# Autodesk Inventor assembly: frame assembly
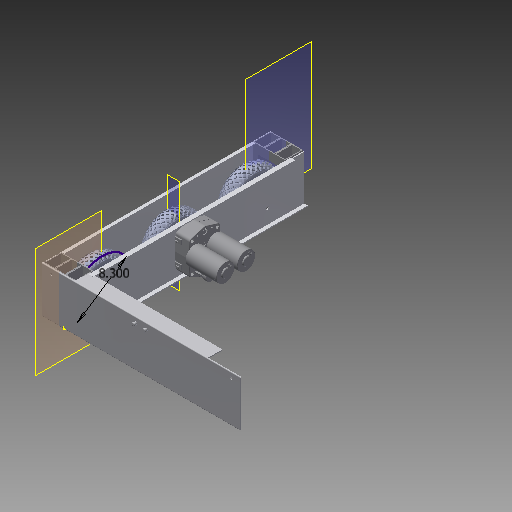
[picture p0: Inventor's stored thumbnail of the model, 512x512]
Saved by Autodesk Inventor 2017 (Build 210142000, 142)
## iProperties
Created: 2019-01-15
Part Number: frame assembly
Document SubType Name: Assembly
Designer: S346795925
Author: S346795925
## Documents named in this file (13)
- P:\frc-season-2019-deep-space-1\Robot\Robot\frame assembly.iam
- P:\frc-season-2019-deep-space-1\Robot\Robot\Frame - outside rail.ipt
- P:\frc-season-2019-deep-space-1\Robot\Robot\am-3936 Aluminum 8IN Pneumatic 500IN Hex Bore Wheel.iam
- P:\frc-season-2019-deep-space-1\Robot\Robot\frame end cap.ipt
- P:\frc-season-2019-deep-space-1\Robot\Robot\Frame - inside rail.ipt
- P:\frc-season-2019-deep-space-1\Robot\Robot\Frame Croner Opposite.ipt
- P:\frc-season-2019-deep-space-1\Robot\Robot\3_CIM_Ball_Shifter_2_Stage_217-3195 (1).iam
- P:\frc-season-2019-deep-space-1\Robot\Robot\OUTERFrame Croner Opposite.ipt
- P:\frc-season-2019-deep-space-1\Robot\Robot\OUTERFrame Croner Opposite_MIR.ipt
- P:\frc-season-2019-deep-space-1\Robot\Robot\Frame Croner Opposite_MIR.ipt
- P:\frc-season-2019-deep-space-1\Robot\Robot\OUTERFrame Croner Opposite_MIR1.ipt
- P:\frc-season-2019-deep-space-1\Robot\Robot\OUTERFrame Croner Opposite_MIR_MIR.ipt
- P:\frc-season-2019-deep-space-1\Robot\Robot\42 tooth HTD Pulley 30mm Wide.iam
## Components (16 placed, 12 different names)
1. Frame - outside rail:1 — Mate:14, Mate:45, Mate:46, Mate:44, Flush:12, Mate:61
2. am-3936 Aluminum 8IN Pneumatic 500IN Hex Bore Wheel:1 [sub-assembly] — Mate:14, Mate:15, Mate:49, Mate:50
3. am-3936 Aluminum 8IN Pneumatic 500IN Hex Bore Wheel:2 [sub-assembly] — Mate:17, Mate:48, Mate:54
4. am-3936 Aluminum 8IN Pneumatic 500IN Hex Bore Wheel:3 [sub-assembly] — Mate:56, Mate:57
5. frame end cap:1 — Mate:59, Flush:12, Mate:60, Angle:1
6. Frame - inside rail:1 — Mate:15, Mate:17, Mate:37, Mate:39, Mate:53, Mate:55, Mate:58
7. 3_CIM_Ball_Shifter_2_Stage_217-3195 (1):1 [sub-assembly] — Mate:37, Mate:39, Angle:1
8. Frame Croner Opposite:2 — Mate:40, Flush:1, Flush:2, Flush:3, Flush:4, Flush:8, Flush:9, Mate:60, Mate:62
9. OUTERFrame Croner Opposite:1 — Mate:40, Flush:1, Flush:2
10. OUTERFrame Croner Opposite_MIR:1 — Flush:8, Flush:9, Mate:59, Mate:61, Mate:62
11. Frame Croner Opposite_MIR:1 — Flush:5, Flush:6, Mate:41, Flush:7, Mate:42, Flush:10, Mate:43, Flush:11, Mate:44
12. OUTERFrame Croner Opposite_MIR1:1 — Flush:5, Flush:6, Mate:41
13. OUTERFrame Croner Opposite_MIR_MIR:1 — Flush:10, Mate:43, Flush:11, Mate:45, Mate:46
14. 42 tooth HTD Pulley 30mm Wide:3 [sub-assembly] — Mate:48, Mate:53, Mate:54
15. 42 tooth HTD Pulley 30mm Wide:4 [sub-assembly] — Mate:49, Mate:50
16. 42 tooth HTD Pulley 30mm Wide:5 [sub-assembly] — Mate:55, Mate:56, Mate:57, Mate:58
## Relationships (38: Mate 25, Flush 12, Angle 1)
- Mate:14: Frame - outside rail:1 ↔ am-3936 Aluminum 8IN Pneumatic 500IN Hex Bore Wheel:1
- Mate:15 (39.37 mm): am-3936 Aluminum 8IN Pneumatic 500IN Hex Bore Wheel:1 ↔ Frame - inside rail:1
- Mate:17 (39.37 mm): am-3936 Aluminum 8IN Pneumatic 500IN Hex Bore Wheel:2 ↔ Frame - inside rail:1
- Mate:37: Frame - inside rail:1 ↔ 3_CIM_Ball_Shifter_2_Stage_217-3195 (1):1
- Mate:39: Frame - inside rail:1 ↔ 3_CIM_Ball_Shifter_2_Stage_217-3195 (1):1
- Mate:40: Frame Croner Opposite:2 ↔ OUTERFrame Croner Opposite:1
- Flush:1: Frame Croner Opposite:2 ↔ OUTERFrame Croner Opposite:1
- Flush:2: Frame Croner Opposite:2 ↔ OUTERFrame Croner Opposite:1
- Flush:3 (19.05 mm): Frame Croner Opposite:2
- Flush:4 (339.725 mm): Frame Croner Opposite:2
- Flush:5: Frame Croner Opposite_MIR:1 ↔ OUTERFrame Croner Opposite_MIR1:1
- Flush:6: Frame Croner Opposite_MIR:1 ↔ OUTERFrame Croner Opposite_MIR1:1
- Mate:41: Frame Croner Opposite_MIR:1 ↔ OUTERFrame Croner Opposite_MIR1:1
- Flush:7 (19.05 mm): Frame Croner Opposite_MIR:1
- Mate:42 (339.725 mm): Frame Croner Opposite_MIR:1
- Flush:8: Frame Croner Opposite:2 ↔ OUTERFrame Croner Opposite_MIR:1
- Flush:9: Frame Croner Opposite:2 ↔ OUTERFrame Croner Opposite_MIR:1
- Flush:10: Frame Croner Opposite_MIR:1 ↔ OUTERFrame Croner Opposite_MIR_MIR:1
- Mate:43: Frame Croner Opposite_MIR:1 ↔ OUTERFrame Croner Opposite_MIR_MIR:1
- Flush:11: Frame Croner Opposite_MIR:1 ↔ OUTERFrame Croner Opposite_MIR_MIR:1
- Mate:44: Frame - outside rail:1 ↔ Frame Croner Opposite_MIR:1
- Mate:45: Frame - outside rail:1 ↔ OUTERFrame Croner Opposite_MIR_MIR:1
- Mate:46: Frame - outside rail:1 ↔ OUTERFrame Croner Opposite_MIR_MIR:1
- Mate:48 (6.35 mm): am-3936 Aluminum 8IN Pneumatic 500IN Hex Bore Wheel:2 ↔ 42 tooth HTD Pulley 30mm Wide:3
- Mate:49: am-3936 Aluminum 8IN Pneumatic 500IN Hex Bore Wheel:1 ↔ 42 tooth HTD Pulley 30mm Wide:4
- Mate:50 (6.35 mm): am-3936 Aluminum 8IN Pneumatic 500IN Hex Bore Wheel:1 ↔ 42 tooth HTD Pulley 30mm Wide:4
- Mate:53: Frame - inside rail:1 ↔ 42 tooth HTD Pulley 30mm Wide:3
- Mate:54: am-3936 Aluminum 8IN Pneumatic 500IN Hex Bore Wheel:2 ↔ 42 tooth HTD Pulley 30mm Wide:3
- Mate:55: Frame - inside rail:1 ↔ 42 tooth HTD Pulley 30mm Wide:5
- Mate:56: am-3936 Aluminum 8IN Pneumatic 500IN Hex Bore Wheel:3 ↔ 42 tooth HTD Pulley 30mm Wide:5
- Mate:57 (6.35 mm): am-3936 Aluminum 8IN Pneumatic 500IN Hex Bore Wheel:3 ↔ 42 tooth HTD Pulley 30mm Wide:5
- Mate:58: Frame - inside rail:1 ↔ 42 tooth HTD Pulley 30mm Wide:5
- Mate:59: frame end cap:1 ↔ OUTERFrame Croner Opposite_MIR:1
- Flush:12: Frame - outside rail:1 ↔ frame end cap:1
- Mate:60: frame end cap:1 ↔ Frame Croner Opposite:2
- Angle:1 (0 deg): frame end cap:1 ↔ 3_CIM_Ball_Shifter_2_Stage_217-3195 (1):1
- Mate:61: Frame - outside rail:1 ↔ OUTERFrame Croner Opposite_MIR:1
- Mate:62: Frame Croner Opposite:2 ↔ OUTERFrame Croner Opposite_MIR:1
